# Autodesk Inventor assembly: Connecting_Plate
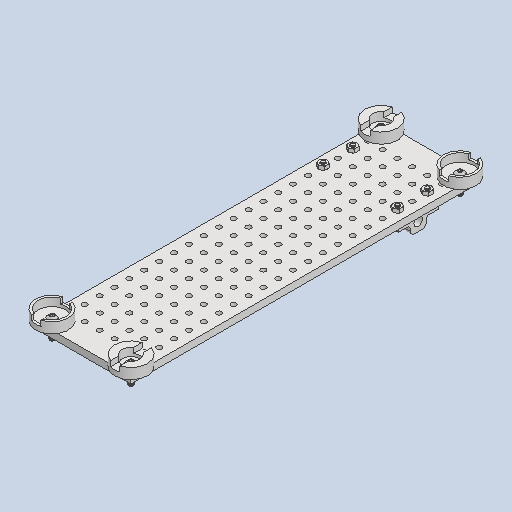
[picture p0: Inventor's stored thumbnail of the model, 512x512]
Saved by Autodesk Inventor 2022.1 (Build 261234020, 234B)
## iProperties
Created: 2021-12-19
Part Number: Connecting_Plate
Document SubType Name: Assembly
Designer: muham
Author: muham
## Documents named in this file (7)
- C:\Users\muham\Desktop\P3_Complete_Revamp\_Cad models\_UpdatedHopperAndSandwichPlate\Hopper_And_Connecting_Plate\Connecting_Plate.iam
- C:\Users\muham\Desktop\P3_Complete_Revamp\_Cad models\_UpdatedHopperAndSandwichPlate\Hopper_And_Connecting_Plate\HopperVR41Y_Base.ipt
- C:\Users\muham\Desktop\P3_Complete_Revamp\_Cad models\_UpdatedHopperAndSandwichPlate\Hopper_And_Connecting_Plate\magnet_spacer2V1.ipt
- C:\Users\muham\Desktop\P3_Complete_Revamp\_Cad models\_UpdatedHopperAndSandwichPlate\Hopper_And_Connecting_Plate\magneticslotV1.ipt
- C:\Users\muham\Desktop\P3_Complete_Revamp\_Cad models\_UpdatedHopperAndSandwichPlate\Hopper_And_Connecting_Plate\M4 x 16mm Machine Screw.ipt
- C:\Users\muham\Desktop\P3_Complete_Revamp\_Cad models\_UpdatedHopperAndSandwichPlate\Hopper_And_Connecting_Plate\M4 Nut.ipt
- C:\Users\muham\Desktop\P3_Complete_Revamp\_Cad models\_UpdatedHopperAndSandwichPlate\Hopper_And_Connecting_Plate\Modular_Single_Axle_V41Y.ipt
## Components (23 placed, 6 different names)
1. HopperVR41Y_Base:1 — Mate:1, Mate:2, Mate:3, Mate:4, Angle:1, Angle:2, Mate:5, Mate:6, Mate:7, Mate:8, Angle:3, Angle:4, Mate:13, Mate:14, Mate:15, Mate:16, Angle:5, Angle:6, Angle:7, Angle:8, Mate:17, Mate:18, Mate:19, Mate:20, Mate:21, Mate:22, Insert:9, Insert:10, Insert:11, Insert:12
2. magnet_spacer2V1:1 — Mate:3, Mate:4, Angle:2, Insert:3
3. magnet_spacer2V1:2 — Mate:1, Mate:2, Angle:1, Insert:1
4. magneticslotV1:1 — Mate:5, Mate:7, Angle:3, Insert:2
5. magneticslotV1:2 — Mate:6, Mate:8, Angle:4, Insert:4
6. M4 x 16mm Machine Screw:1 — Insert:1, Mate:9
7. M4 x 16mm Machine Screw:2 — Insert:2, Mate:10
8. M4 x 16mm Machine Screw:3 — Insert:4, Mate:11
9. M4 x 16mm Machine Screw:4 — Insert:3, Mate:12
10. M4 Nut:1 — Mate:9, Mate:16, Angle:8
11. M4 Nut:2 — Mate:10, Mate:15, Angle:7
12. M4 Nut:3 — Mate:11, Mate:13, Angle:6
13. M4 Nut:4 — Mate:12, Mate:14, Angle:5
14. Modular_Single_Axle_V41Y:1 — Mate:17, Mate:18, Mate:19, Insert:7, Insert:8
15. Modular_Single_Axle_V41Y:2 — Mate:20, Mate:21, Mate:22, Insert:5, Insert:6
16. M4 x 16mm Machine Screw:5 — Insert:5
17. M4 x 16mm Machine Screw:6 — Insert:6
18. M4 x 16mm Machine Screw:7 — Insert:7
19. M4 x 16mm Machine Screw:8 — Insert:8
20. M4 Nut:5 — Insert:9
21. M4 Nut:6 — Insert:10
22. M4 Nut:7 — Insert:11
23. M4 Nut:8 — Insert:12
## Relationships (42: Mate 22, Insert 12, Angle 8)
- Mate:1: HopperVR41Y_Base:1 ↔ magnet_spacer2V1:2
- Mate:2: HopperVR41Y_Base:1 ↔ magnet_spacer2V1:2
- Mate:3: HopperVR41Y_Base:1 ↔ magnet_spacer2V1:1
- Mate:4: HopperVR41Y_Base:1 ↔ magnet_spacer2V1:1
- Angle:1 (90 deg): HopperVR41Y_Base:1 ↔ magnet_spacer2V1:2
- Angle:2 (90 deg): HopperVR41Y_Base:1 ↔ magnet_spacer2V1:1
- Mate:5: HopperVR41Y_Base:1 ↔ magneticslotV1:1
- Mate:6: HopperVR41Y_Base:1 ↔ magneticslotV1:2
- Mate:7: HopperVR41Y_Base:1 ↔ magneticslotV1:1
- Mate:8: HopperVR41Y_Base:1 ↔ magneticslotV1:2
- Angle:3 (0 deg): HopperVR41Y_Base:1 ↔ magneticslotV1:1
- Angle:4 (0 deg): HopperVR41Y_Base:1 ↔ magneticslotV1:2
- Insert:1: magnet_spacer2V1:2 ↔ M4 x 16mm Machine Screw:1
- Insert:2: magneticslotV1:1 ↔ M4 x 16mm Machine Screw:2
- Insert:3: magnet_spacer2V1:1 ↔ M4 x 16mm Machine Screw:4
- Insert:4: magneticslotV1:2 ↔ M4 x 16mm Machine Screw:3
- Mate:9: M4 x 16mm Machine Screw:1 ↔ M4 Nut:1
- Mate:10: M4 x 16mm Machine Screw:2 ↔ M4 Nut:2
- Mate:11: M4 x 16mm Machine Screw:3 ↔ M4 Nut:3
- Mate:12: M4 x 16mm Machine Screw:4 ↔ M4 Nut:4
- Mate:13: HopperVR41Y_Base:1 ↔ M4 Nut:3
- Mate:14: HopperVR41Y_Base:1 ↔ M4 Nut:4
- Mate:15: HopperVR41Y_Base:1 ↔ M4 Nut:2
- Mate:16: HopperVR41Y_Base:1 ↔ M4 Nut:1
- Angle:5 (0 deg): HopperVR41Y_Base:1 ↔ M4 Nut:4
- Angle:6 (0 deg): HopperVR41Y_Base:1 ↔ M4 Nut:3
- Angle:7 (0 deg): HopperVR41Y_Base:1 ↔ M4 Nut:2
- Angle:8 (0 deg): HopperVR41Y_Base:1 ↔ M4 Nut:1
- Mate:17: HopperVR41Y_Base:1 ↔ Modular_Single_Axle_V41Y:1
- Mate:18: HopperVR41Y_Base:1 ↔ Modular_Single_Axle_V41Y:1
- Mate:19: HopperVR41Y_Base:1 ↔ Modular_Single_Axle_V41Y:1
- Mate:20: HopperVR41Y_Base:1 ↔ Modular_Single_Axle_V41Y:2
- Mate:21: HopperVR41Y_Base:1 ↔ Modular_Single_Axle_V41Y:2
- Mate:22: HopperVR41Y_Base:1 ↔ Modular_Single_Axle_V41Y:2
- Insert:5: Modular_Single_Axle_V41Y:2 ↔ M4 x 16mm Machine Screw:5
- Insert:6: Modular_Single_Axle_V41Y:2 ↔ M4 x 16mm Machine Screw:6
- Insert:7: Modular_Single_Axle_V41Y:1 ↔ M4 x 16mm Machine Screw:7
- Insert:8: Modular_Single_Axle_V41Y:1 ↔ M4 x 16mm Machine Screw:8
- Insert:9: HopperVR41Y_Base:1 ↔ M4 Nut:5
- Insert:10: HopperVR41Y_Base:1 ↔ M4 Nut:6
- Insert:11: HopperVR41Y_Base:1 ↔ M4 Nut:7
- Insert:12: HopperVR41Y_Base:1 ↔ M4 Nut:8
